# Autodesk Inventor assembly: Конструкция
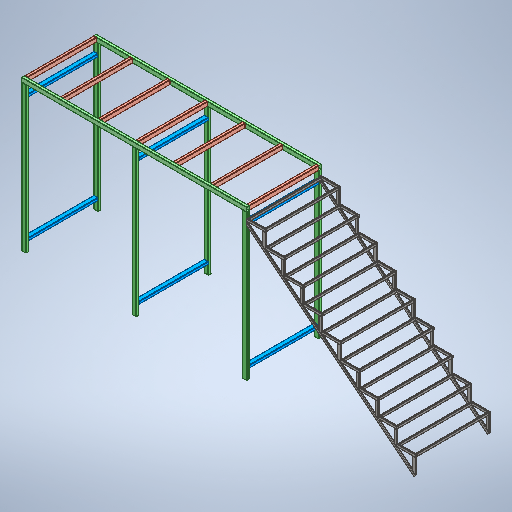
[picture p0: Inventor's stored thumbnail of the model, 512x512]
Saved by Autodesk Inventor 2025 (Build 290162010, 162A)
## iProperties
Created: 2024-08-28
Part Number: Конструкция
Document SubType Name: Assembly
Designer: pokla
Author: pokla
## Documents named in this file (5)
- C:\Users\pokla\Documents\Inventor\BSH_Beshkino_bio_tank\Конструкция.iam
- C:\Users\pokla\Documents\Inventor\BSH_Beshkino_bio_tank\лестница\Перегородка\ASY NDM 11.030 перегородка рама 2 горизонт.iam
- C:\Users\pokla\Documents\Inventor\BSH_Beshkino_bio_tank\лестница\Перегородка\ASY NDM 11.050 перегородка рама 2 вертикал.iam
- C:\Users\pokla\Documents\Inventor\BSH_Beshkino_bio_tank\Assembly5.iam
- C:\Users\pokla\Documents\Inventor\BSH_Beshkino_bio_tank\Тетива.iam
## Components (15 placed, 4 different names)
1. ASY NDM 11.030 перегородка рама 2 горизонт:1 [sub-assembly] — Flush:2
2. ASY NDM 11.050 перегородка рама 2 вертикал:1 [sub-assembly] — Mate:7, Mate:8
3. ASY NDM 11.050 перегородка рама 2 вертикал:2 [sub-assembly]
4. ASY NDM 11.050 перегородка рама 2 вертикал:3 [sub-assembly]
5. Тетива:2 [sub-assembly] — Mate:4, Flush:4, Mate:7
6. Тетива:3 [sub-assembly] — Mate:6, Flush:8, Mate:8
7. Assembly5:1 [sub-assembly] — Flush:2
8. Assembly5:2 [sub-assembly]
9. Assembly5:3 [sub-assembly]
10. Assembly5:4 [sub-assembly]
11. Assembly5:5 [sub-assembly]
12. Assembly5:6 [sub-assembly]
13. Assembly5:7 [sub-assembly]
14. Assembly5:8 [sub-assembly]
15. Assembly5:9 [sub-assembly] — Mate:4, Flush:4, Mate:6, Flush:8
## Component patterns: (9 elements, first: Assembly5:1)
## Relationships (12: Mate 5, Flush 4, WeldJoint 3)
- [WeldJoint]: ASY NDM 11.030 перегородка рама 2 горизонт:1 ↔ ASY NDM 11.050 перегородка рама 2 вертикал:1
- [WeldJoint]: ASY NDM 11.030 перегородка рама 2 горизонт:1 ↔ ASY NDM 11.050 перегородка рама 2 вертикал:3
- [WeldJoint]: ASY NDM 11.030 перегородка рама 2 горизонт:1 ↔ ASY NDM 11.050 перегородка рама 2 вертикал:2
- [Flush]: ASY NDM 11.030 перегородка рама 2 горизонт:1 ↔ Assembly5:1
- [Mate]: ASY NDM 11.030 перегородка рама 2 горизонт:1 ↔ Assembly5:1
- Flush:2 (129.013 mm): ASY NDM 11.030 перегородка рама 2 горизонт:1 ↔ Assembly5:1
- Mate:4: Тетива:2 ↔ Assembly5:9
- Flush:4: Тетива:2 ↔ Assembly5:9
- Mate:6: Тетива:3 ↔ Assembly5:9
- Flush:8: Тетива:3 ↔ Assembly5:9
- Mate:7: ASY NDM 11.050 перегородка рама 2 вертикал:1 ↔ Тетива:2
- Mate:8: ASY NDM 11.050 перегородка рама 2 вертикал:1 ↔ Тетива:3
